# Autodesk Inventor assembly: 50_Assembly_ETL_Mould
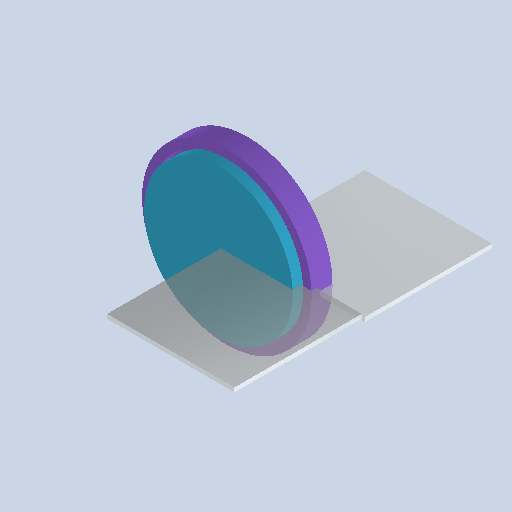
[picture p0: Inventor's stored thumbnail of the model, 512x512]
Saved by Autodesk Inventor 2022.3 (Build 263350000, 350)
## iProperties
Created: 2022-01-02
Part Number: 50_Assembly_ETL_Mould
Document SubType Name: Assembly
Designer: diederichbenedict
Author: diederichbenedict
## Documents named in this file (5)
- G:\My Drive\ASP - M.Sc. Photonics\Practical Modules\MODULE 4 - Master Thesis\2.Experiments\Modules\11.Reference_Mirror_Module\Reference_Mirror_with_UC2-VCA_Module\50_Assembly_ETL_Mould.iam
- G:\My Drive\ASP - M.Sc. Photonics\Practical Modules\MODULE 4 - Master Thesis\2.Experiments\Modules\11.Reference_Mirror_Module\Reference_Mirror_with_UC2-VCA_Module\50_ETL_Membrane_v0.ipt
- G:\My Drive\ASP - M.Sc. Photonics\Practical Modules\MODULE 4 - Master Thesis\2.Experiments\Modules\11.Reference_Mirror_Module\Reference_Mirror_with_UC2-VCA_Module\50_ETL_Membrane_Mould_Lower_v0.ipt
- G:\My Drive\ASP - M.Sc. Photonics\Practical Modules\MODULE 4 - Master Thesis\2.Experiments\Modules\11.Reference_Mirror_Module\Reference_Mirror_with_UC2-VCA_Module\50_ETL_Membrane_Mould_Upper_v0.ipt
- G:\My Drive\ASP - M.Sc. Photonics\Practical Modules\MODULE 4 - Master Thesis\2.Experiments\Modules\11.Reference_Mirror_Module\Reference_Mirror_with_UC2-VCA_Module\00_Mirror_30x30.ipt
## Components (5 placed, 4 different names)
1. 50_ETL_Membrane_v0:1 — Passend:3
2. 50_ETL_Membrane_Mould_Lower_v0:1 — Passend:2, Einfügen:1
3. 50_ETL_Membrane_Mould_Upper_v0:1 — Passend:1, Einfügen:2
4. 00_Mirror_30x30:1 — Einfügen:1
5. 00_Mirror_30x30:2 — Einfügen:2
## Relationships (7: Mate 3, Flush 2, Insert 2)
- [Flush]: 50_ETL_Membrane_v0:1 ↔ 50_ETL_Membrane_Mould_Lower_v0:1
- [Flush]: 50_ETL_Membrane_Mould_Lower_v0:1 ↔ 50_ETL_Membrane_Mould_Upper_v0:1
- Passend:1 [Mate]: 50_ETL_Membrane_Mould_Upper_v0:1
- Passend:2 [Mate]: 50_ETL_Membrane_Mould_Lower_v0:1
- Passend:3 [Mate]: 50_ETL_Membrane_v0:1
- Einfügen:1 [Insert]: 50_ETL_Membrane_Mould_Lower_v0:1 ↔ 00_Mirror_30x30:1
- Einfügen:2 [Insert]: 50_ETL_Membrane_Mould_Upper_v0:1 ↔ 00_Mirror_30x30:2
